# Autodesk Inventor assembly: ParticleLauncherwCollector
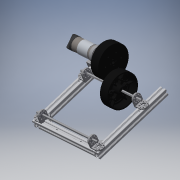
[picture p0: Inventor's stored thumbnail of the model, 180x180]
Saved by Autodesk Inventor 2016 (Build 200138000, 138)
## iProperties
Created: 2016-10-12
Part Number: ParticleLauncherwCollector
Document SubType Name: Assembly
Designer: Delta
Author: Delta
## Documents named in this file (12)
- C:\Robotics\CAD\2016-17_CAD\ParticleLauncherwCollector.iam
- C:\Robotics\CAD\COTSParts\Actobotics\555 parts\555116.ipt
- C:\Robotics\CAD\COTSParts\Actobotics\am-3102NeveRest20 (1).ipt
- C:\Robotics\CAD\COTSParts\Actobotics\634 parts\634088.ipt
- C:\Robotics\CAD\COTSParts\Wheels\4in Wheel Intergreated Hub 8mm Rev2.ipt
- C:\Robotics\CAD\COTSParts\Bosch Extrusion\Bosch 20x20 9 in.ipt
- C:\Robotics\CAD\COTSParts\Bearings - AndyMark\Bearing 250 ID 500 OD flanged.ipt
- C:\Robotics\CAD\COTSParts\Actobotics\545 parts\545400.ipt
- C:\Robotics\CAD\COTSParts\Bosch Extrusion\6mm block nut M4.ipt
- C:\Robotics\CAD\COTSParts\Actobotics\585 parts\585494.ipt
- C:\Robotics\CAD\COTSParts\Bosch Extrusion\Bosch 20x20 - 7.184 Part.Shoot.ipt
- C:\Robotics\CAD\COTSParts\Bosch Extrusion\Gusset 20x20 w screws.ipt
## Components (30 placed, 11 different names)
1. 555116:1 — Insert:15, Insert:35, Insert:36
2. am-3102NeveRest20 (1):1 — Insert:15, Insert:34
3. 634088:1 — Insert:17, Insert:42, Insert:57
4. 4in Wheel Intergreated Hub 8mm Rev2:1 — Insert:17
5. 4in Wheel Intergreated Hub 8mm Rev2:2 — Insert:34
6. Bosch 20x20 9 in:1 — Mate:7, Mate:8, Mate:9, Mate:10, Flush:8, Flush:9, Mate:16, Mate:17, Mate:18, Mate:19, Flush:10, Flush:11, Flush:12, Mate:20, Mate:21, Mate:22, Mate:23, Flush:13, Mate:28, Mate:29, Flush:15
7. Bosch 20x20 9 in:2 — Mate:11, Mate:12, Mate:13, Mate:14, Flush:8, Flush:9, Flush:11, Flush:12, Mate:24, Mate:25, Mate:26, Mate:27, Flush:14, Mate:33, Mate:36, Mate:37
8. Bearing 250 ID 500 OD flanged:2 — Insert:41, Insert:42
9. Bearing 250 ID 500 OD flanged:3 — Insert:48, Insert:57
10. 545400:1 — Insert:45, Insert:46, Insert:48
11. 545400:2 — Insert:39, Insert:40, Insert:41
12. 6mm block nut M4:1 — Mate:16, Mate:17, Insert:44
13. 6mm block nut M4:2 — Mate:18, Mate:19, Flush:10, Insert:43
14. 6mm block nut M4:4 — Mate:7, Mate:8, Insert:45
15. 6mm block nut M4:5 — Mate:9, Mate:10, Insert:46
16. 6mm block nut M4:6 — Mate:13, Mate:14, Insert:39
17. 6mm block nut M4:7 — Mate:11, Mate:12, Insert:40
18. 585494:2 — Insert:35, Insert:36, Insert:43, Insert:44
19. 6mm block nut M4:8 — Mate:20, Mate:21, Insert:52
20. 6mm block nut M4:9 — Mate:26, Mate:27, Insert:49, Flush:14
21. 6mm block nut M4:10 — Mate:24, Mate:25, Insert:50
22. 6mm block nut M4:11 — Mate:22, Mate:23, Insert:51, Flush:13
23. 634088:2 — Insert:53
24. 545400:3 — Insert:49, Insert:50, Insert:55
25. 545400:4 — Insert:51, Insert:52, Insert:56
26. Bearing 250 ID 500 OD flanged:4 — Insert:56
27. Bearing 250 ID 500 OD flanged:5 — Insert:53, Insert:55
28. Bosch 20x20 - 7.184 Part.Shoot:1 — Mate:30, Mate:31, Mate:33, Mate:34, Mate:35, Flush:15
29. Gusset 20x20 w screws:1 — Mate:28, Mate:29, Mate:30, Mate:31
30. Gusset 20x20 w screws:2 — Mate:34, Mate:35, Mate:36, Mate:37
## Relationships (59: Mate 29, Insert 22, Flush 8)
- Insert:15 (-9.525 mm): 555116:1 ↔ am-3102NeveRest20 (1):1
- Insert:17 (63.5 mm): 634088:1 ↔ 4in Wheel Intergreated Hub 8mm Rev2:1
- Mate:7: Bosch 20x20 9 in:1 ↔ 6mm block nut M4:4
- Mate:8: Bosch 20x20 9 in:1 ↔ 6mm block nut M4:4
- Mate:9: Bosch 20x20 9 in:1 ↔ 6mm block nut M4:5
- Mate:10: Bosch 20x20 9 in:1 ↔ 6mm block nut M4:5
- Mate:11: Bosch 20x20 9 in:2 ↔ 6mm block nut M4:7
- Mate:12: Bosch 20x20 9 in:2 ↔ 6mm block nut M4:7
- Mate:13: Bosch 20x20 9 in:2 ↔ 6mm block nut M4:6
- Mate:14: Bosch 20x20 9 in:2 ↔ 6mm block nut M4:6
- Flush:8: Bosch 20x20 9 in:1 ↔ Bosch 20x20 9 in:2
- Flush:9: Bosch 20x20 9 in:1 ↔ Bosch 20x20 9 in:2
- Insert:34 (-10.16 mm): am-3102NeveRest20 (1):1 ↔ 4in Wheel Intergreated Hub 8mm Rev2:2
- Insert:35: 555116:1 ↔ 585494:2
- Insert:36: 555116:1 ↔ 585494:2
- Mate:16: Bosch 20x20 9 in:1 ↔ 6mm block nut M4:1
- Mate:17: Bosch 20x20 9 in:1 ↔ 6mm block nut M4:1
- Mate:18: Bosch 20x20 9 in:1 ↔ 6mm block nut M4:2
- Mate:19: Bosch 20x20 9 in:1 ↔ 6mm block nut M4:2
- Flush:10: Bosch 20x20 9 in:1 ↔ 6mm block nut M4:2
- Insert:39: 545400:2 ↔ 6mm block nut M4:6
- Insert:40: 545400:2 ↔ 6mm block nut M4:7
- Insert:41: Bearing 250 ID 500 OD flanged:2 ↔ 545400:2
- Insert:42 (20.32 mm): 634088:1 ↔ Bearing 250 ID 500 OD flanged:2
- Insert:43: 6mm block nut M4:2 ↔ 585494:2
- Insert:44: 6mm block nut M4:1 ↔ 585494:2
- Insert:45: 545400:1 ↔ 6mm block nut M4:4
- Insert:46: 545400:1 ↔ 6mm block nut M4:5
- Flush:11: Bosch 20x20 9 in:1 ↔ Bosch 20x20 9 in:2
- Flush:12: Bosch 20x20 9 in:1 ↔ Bosch 20x20 9 in:2
- Insert:48: Bearing 250 ID 500 OD flanged:3 ↔ 545400:1
- Mate:20: Bosch 20x20 9 in:1 ↔ 6mm block nut M4:8
- Mate:21: Bosch 20x20 9 in:1 ↔ 6mm block nut M4:8
- Mate:22: Bosch 20x20 9 in:1 ↔ 6mm block nut M4:11
- Mate:23: Bosch 20x20 9 in:1 ↔ 6mm block nut M4:11
- Mate:24: Bosch 20x20 9 in:2 ↔ 6mm block nut M4:10
- Mate:25: Bosch 20x20 9 in:2 ↔ 6mm block nut M4:10
- Mate:26: Bosch 20x20 9 in:2 ↔ 6mm block nut M4:9
- Mate:27: Bosch 20x20 9 in:2 ↔ 6mm block nut M4:9
- Insert:49: 6mm block nut M4:9 ↔ 545400:3
- Insert:50: 6mm block nut M4:10 ↔ 545400:3
- Insert:51: 6mm block nut M4:11 ↔ 545400:4
- Insert:52: 6mm block nut M4:8 ↔ 545400:4
- Flush:13: Bosch 20x20 9 in:1 ↔ 6mm block nut M4:11
- Flush:14: Bosch 20x20 9 in:2 ↔ 6mm block nut M4:9
- Insert:53 (20.32 mm): 634088:2 ↔ Bearing 250 ID 500 OD flanged:5
- Insert:55: 545400:3 ↔ Bearing 250 ID 500 OD flanged:5
- Insert:56: 545400:4 ↔ Bearing 250 ID 500 OD flanged:4
- Insert:57 (20.32 mm): 634088:1 ↔ Bearing 250 ID 500 OD flanged:3
- Mate:28: Bosch 20x20 9 in:1 ↔ Gusset 20x20 w screws:1
- Mate:29: Bosch 20x20 9 in:1 ↔ Gusset 20x20 w screws:1
- Mate:30: Bosch 20x20 - 7.184 Part.Shoot:1 ↔ Gusset 20x20 w screws:1
- Mate:31: Bosch 20x20 - 7.184 Part.Shoot:1 ↔ Gusset 20x20 w screws:1
- Mate:33: Bosch 20x20 9 in:2 ↔ Bosch 20x20 - 7.184 Part.Shoot:1
- Mate:34: Bosch 20x20 - 7.184 Part.Shoot:1 ↔ Gusset 20x20 w screws:2
- Mate:35: Bosch 20x20 - 7.184 Part.Shoot:1 ↔ Gusset 20x20 w screws:2
- Mate:36: Bosch 20x20 9 in:2 ↔ Gusset 20x20 w screws:2
- Mate:37: Bosch 20x20 9 in:2 ↔ Gusset 20x20 w screws:2
- Flush:15: Bosch 20x20 9 in:1 ↔ Bosch 20x20 - 7.184 Part.Shoot:1
